# Autodesk Inventor assembly: Gen 2.0 Robot
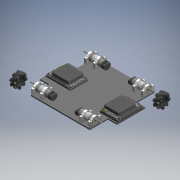
[picture p0: Inventor's stored thumbnail of the model, 180x180]
Saved by Autodesk Inventor 2019 (Build 230136000, 136)
## iProperties
Part Number: Gen 2.0 Robot
Document SubType Name: Assembly
Designer: Delta
Author: Delta
## Documents named in this file (6)
- C:\Robotics\2019-20_CAD\Drive Train\Gen 2.0 Robot.iam
- C:\Robotics\2019-20_CAD\Drive Train\Gen 2.0 rev mecanums base plate.ipt
- C:\Robotics\COTSParts\Motors\am-3102NeveRest20 (1).ipt
- C:\Robotics\COTSParts\Tetrix\tetrix-motor-mounts-1.snapshot.1\Tetrex 2pc motor mount.ipt
- C:\Robotics\COTSParts\Rev\REV-31-1153RevHub.ipt
- C:\Robotics\COTSParts\Rev\REV-41-1656MecanumWheel.iam
## Components (17 placed, 5 different names)
1. Gen 2.0 rev mecanums base plate:1 — Mate:1, Flush:1, Flush:2, Flush:3, Mate:2, Flush:6, Flush:7, Mate:4, Flush:8, Mate:5, Flush:11, Flush:12, Mate:7, Flush:13, Mate:8, Flush:16, Mate:10, Flush:17, Flush:18, Mate:11, Mate:13, Mate:14, Mate:15, Mate:16, Mate:17
2. am-3102NeveRest20 (1):1 — Mate:12, Flush:19, Flush:20
3. am-3102NeveRest20 (1):2 — Mate:9, Flush:14, Flush:15
4. am-3102NeveRest20 (1):3 — Mate:3, Flush:4, Flush:5
5. am-3102NeveRest20 (1):4 — Mate:6, Flush:9, Flush:10
6. Tetrex 2pc motor mount:1 — Flush:3, Mate:2, Flush:5
7. Tetrex 2pc motor mount:2 — Mate:1, Flush:1, Flush:2, Mate:3, Flush:4
8. Tetrex 2pc motor mount:3 — Flush:13, Mate:8, Flush:15
9. Tetrex 2pc motor mount:4 — Flush:11, Flush:12, Mate:7, Mate:9, Flush:14
10. Tetrex 2pc motor mount:5 — Flush:16, Mate:10, Flush:17, Mate:12, Flush:19
11. Tetrex 2pc motor mount:6 — Flush:18, Mate:11, Flush:20
12. Tetrex 2pc motor mount:7 — Flush:8, Mate:5, Flush:10
13. Tetrex 2pc motor mount:8 — Flush:6, Flush:7, Mate:4, Mate:6, Flush:9
14. REV-31-1153RevHub:1 — Mate:13, Mate:14, Mate:15
15. REV-31-1153RevHub:2 — Mate:16, Mate:17
16. REV-41-1656MecanumWheel:1 [sub-assembly]
17. REV-41-1656MecanumWheel:2 [sub-assembly]
## Relationships (37: Flush 20, Mate 17)
- Mate:1: Gen 2.0 rev mecanums base plate:1 ↔ Tetrex 2pc motor mount:2
- Flush:1: Gen 2.0 rev mecanums base plate:1 ↔ Tetrex 2pc motor mount:2
- Flush:2: Gen 2.0 rev mecanums base plate:1 ↔ Tetrex 2pc motor mount:2
- Flush:3: Gen 2.0 rev mecanums base plate:1 ↔ Tetrex 2pc motor mount:1
- Mate:2: Gen 2.0 rev mecanums base plate:1 ↔ Tetrex 2pc motor mount:1
- Mate:3: am-3102NeveRest20 (1):3 ↔ Tetrex 2pc motor mount:2
- Flush:4: am-3102NeveRest20 (1):3 ↔ Tetrex 2pc motor mount:2
- Flush:5: am-3102NeveRest20 (1):3 ↔ Tetrex 2pc motor mount:1
- Flush:6: Gen 2.0 rev mecanums base plate:1 ↔ Tetrex 2pc motor mount:8
- Flush:7: Gen 2.0 rev mecanums base plate:1 ↔ Tetrex 2pc motor mount:8
- Mate:4: Gen 2.0 rev mecanums base plate:1 ↔ Tetrex 2pc motor mount:8
- Flush:8: Gen 2.0 rev mecanums base plate:1 ↔ Tetrex 2pc motor mount:7
- Mate:5: Gen 2.0 rev mecanums base plate:1 ↔ Tetrex 2pc motor mount:7
- Mate:6: am-3102NeveRest20 (1):4 ↔ Tetrex 2pc motor mount:8
- Flush:9: am-3102NeveRest20 (1):4 ↔ Tetrex 2pc motor mount:8
- Flush:10: am-3102NeveRest20 (1):4 ↔ Tetrex 2pc motor mount:7
- Flush:11: Gen 2.0 rev mecanums base plate:1 ↔ Tetrex 2pc motor mount:4
- Flush:12: Gen 2.0 rev mecanums base plate:1 ↔ Tetrex 2pc motor mount:4
- Mate:7: Gen 2.0 rev mecanums base plate:1 ↔ Tetrex 2pc motor mount:4
- Flush:13: Gen 2.0 rev mecanums base plate:1 ↔ Tetrex 2pc motor mount:3
- Mate:8: Gen 2.0 rev mecanums base plate:1 ↔ Tetrex 2pc motor mount:3
- Mate:9: am-3102NeveRest20 (1):2 ↔ Tetrex 2pc motor mount:4
- Flush:14: am-3102NeveRest20 (1):2 ↔ Tetrex 2pc motor mount:4
- Flush:15: am-3102NeveRest20 (1):2 ↔ Tetrex 2pc motor mount:3
- Flush:16: Gen 2.0 rev mecanums base plate:1 ↔ Tetrex 2pc motor mount:5
- Mate:10: Gen 2.0 rev mecanums base plate:1 ↔ Tetrex 2pc motor mount:5
- Flush:17: Gen 2.0 rev mecanums base plate:1 ↔ Tetrex 2pc motor mount:5
- Flush:18: Gen 2.0 rev mecanums base plate:1 ↔ Tetrex 2pc motor mount:6
- Mate:11: Gen 2.0 rev mecanums base plate:1 ↔ Tetrex 2pc motor mount:6
- Mate:12: am-3102NeveRest20 (1):1 ↔ Tetrex 2pc motor mount:5
- Flush:19: am-3102NeveRest20 (1):1 ↔ Tetrex 2pc motor mount:5
- Flush:20: am-3102NeveRest20 (1):1 ↔ Tetrex 2pc motor mount:6
- Mate:13: Gen 2.0 rev mecanums base plate:1 ↔ REV-31-1153RevHub:1
- Mate:14: Gen 2.0 rev mecanums base plate:1 ↔ REV-31-1153RevHub:1
- Mate:15 (-10.05 mm): Gen 2.0 rev mecanums base plate:1 ↔ REV-31-1153RevHub:1
- Mate:16: Gen 2.0 rev mecanums base plate:1 ↔ REV-31-1153RevHub:2
- Mate:17 (-27.8765 mm): Gen 2.0 rev mecanums base plate:1 ↔ REV-31-1153RevHub:2
